# Autodesk Inventor assembly: hip_joint_fix_washer_10mm_Set
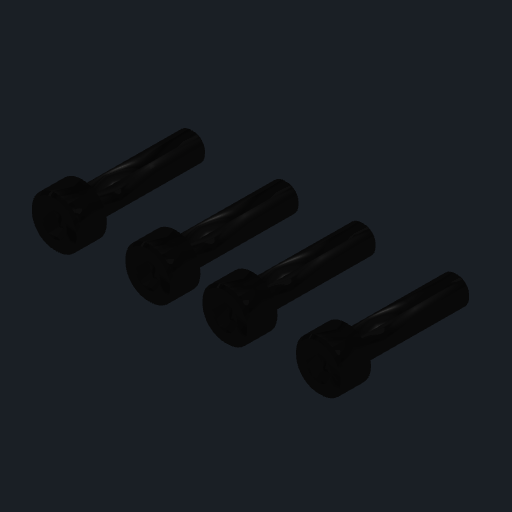
[picture p0: Inventor's stored thumbnail of the model, 512x512]
Saved by Autodesk Inventor 2024.3 (Build 283343000, 343)
## iProperties
Created: 2024-01-28
Part Number: hip_joint_fix_washer_10mm_Set
Document SubType Name: Assembly
Designer: 김대겸
Author: 김대겸
## Documents named in this file (2)
- C:\Users\ASUS\Desktop\test\Screw_Set\hip_joint_fix_washer_10mm_Set.iam
- C:\Users\ASUS\Desktop\test\v1_Frame\MISUMI\CSH-ST-M2_5-10.ipt
## Components (4 placed, 1 different names)
1. CSH-ST-M2_5-10:1 — 플러쉬:3, 메이트:3, 플러쉬:6
2. CSH-ST-M2_5-10:2 — 플러쉬:1, 메이트:1, 플러쉬:4
3. CSH-ST-M2_5-10:3 — 플러쉬:2, 플러쉬:3, 메이트:2, 메이트:3, 플러쉬:5, 플러쉬:6
4. CSH-ST-M2_5-10:4 — 플러쉬:1, 플러쉬:2, 메이트:1, 메이트:2, 플러쉬:4, 플러쉬:5
## Relationships (9: Flush 6, Mate 3)
- 플러쉬:1 [Flush]: CSH-ST-M2_5-10:2 ↔ CSH-ST-M2_5-10:4
- 플러쉬:2 [Flush]: CSH-ST-M2_5-10:3 ↔ CSH-ST-M2_5-10:4
- 플러쉬:3 [Flush]: CSH-ST-M2_5-10:1 ↔ CSH-ST-M2_5-10:3
- 메이트:1 [Mate] (-8.5 mm): CSH-ST-M2_5-10:2 ↔ CSH-ST-M2_5-10:4
- 메이트:2 [Mate] (7 mm): CSH-ST-M2_5-10:3 ↔ CSH-ST-M2_5-10:4
- 메이트:3 [Mate] (8.5 mm): CSH-ST-M2_5-10:1 ↔ CSH-ST-M2_5-10:3
- 플러쉬:4 [Flush]: CSH-ST-M2_5-10:2 ↔ CSH-ST-M2_5-10:4
- 플러쉬:5 [Flush]: CSH-ST-M2_5-10:3 ↔ CSH-ST-M2_5-10:4
- 플러쉬:6 [Flush]: CSH-ST-M2_5-10:1 ↔ CSH-ST-M2_5-10:3
